# Autodesk Inventor assembly: вертикальный ЗАХВАТ
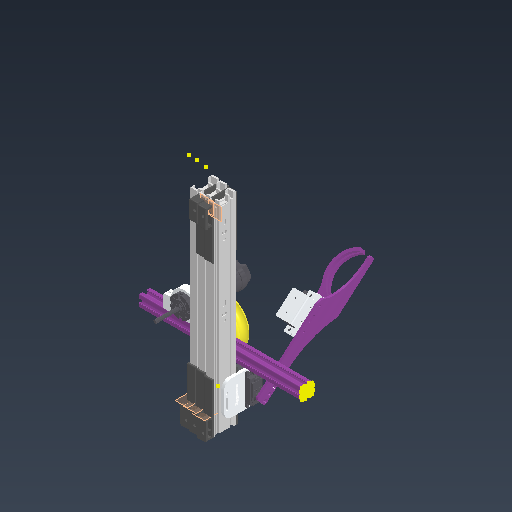
[picture p0: Inventor's stored thumbnail of the model, 512x512]
Saved by Autodesk Inventor 2025 (Build 290162000, 162)
## iProperties
Created: 2025-01-28
Part Number: вертикальный ЗАХВАТ
Document SubType Name: Assembly
Designer: GameHD
Author: GameHD
## Documents named in this file (12)
- C:\Users\GameHD\Desktop\phantom 16950\вертикальный ЗАХВАТ.iam
- C:\Users\GameHD\Desktop\phantom 16950\2000-0025-0002\2000-0025-0002_MIR1.ipt
- C:\Users\GameHD\Desktop\phantom 16950\клешня сос_MIR.ipt
- C:\Users\GameHD\Desktop\phantom 16950\39060_txm-standard servo bracket\39060_txm-standard servo bracket_MIR.ipt
- C:\Users\GameHD\Desktop\phantom 16950\Клешни с фиксатором\Клешни с фиксатором_MIR_MIR.ipt
- C:\Users\GameHD\Desktop\phantom 16950\профиль каркас ГОРИЗОНТ пенпер.ipt
- C:\Users\GameHD\Desktop\phantom 16950\35 напр.iam
- C:\Users\GameHD\Desktop\phantom 16950\39089_txm-motormount\39089_txm-motormount.ipt
- C:\Users\GameHD\Desktop\phantom 16950\REV-41-1211\REV-41-1211.ipt
- C:\Users\GameHD\Desktop\phantom 16950\пластинка для серв.ipt
- C:\Users\GameHD\Desktop\phantom 16950\katushechka_pushechka\katushechka_pushechka_CPY.ipt
- C:\Users\GameHD\Desktop\phantom 16950\katushechka_pushechka 2\katushechka_pushechka 2_CPY.ipt
## Components (12 placed, 11 different names)
1. профиль каркас ГОРИЗОНТ пенпер:1
2. 2000-0025-0002_MIR1:1
3. клешня сос_MIR:1
4. 39060_txm-standard servo bracket_MIR:1
5. 2000-0025-0002_MIR1:2
6. Клешни с фиксатором_MIR_MIR:1
7. 35 напр:1 [sub-assembly]
8. 39089_txm-motormount:1
9. REV-41-1211:1
10. пластинка для серв:1
11. katushechka_pushechka_CPY:1 — Совмещение:16, Совмещение:17
12. katushechka_pushechka 2_CPY:1 — Совмещение:16, Совмещение:17
## Relationships (19: Mate 14, Flush 5)
- [Flush] (-90 mm): клешня сос_MIR:1 ↔ 39060_txm-standard servo bracket_MIR:1
- [Flush]: клешня сос_MIR:1 ↔ 39060_txm-standard servo bracket_MIR:1
- [Mate]: клешня сос_MIR:1 ↔ 39060_txm-standard servo bracket_MIR:1
- [Mate] (4 mm): 39060_txm-standard servo bracket_MIR:1 ↔ 2000-0025-0002_MIR1:2
- [Flush] (2.5 mm): 39060_txm-standard servo bracket_MIR:1 ↔ 2000-0025-0002_MIR1:2
- [Mate]: 39060_txm-standard servo bracket_MIR:1 ↔ 2000-0025-0002_MIR1:2
- [Mate] (7 mm): клешня сос_MIR:1 ↔ Клешни с фиксатором_MIR_MIR:1
- [Mate]: 2000-0025-0002_MIR1:2 ↔ Клешни с фиксатором_MIR_MIR:1
- [Mate]: 2000-0025-0002_MIR1:2 ↔ Клешни с фиксатором_MIR_MIR:1
- [Mate]: профиль каркас ГОРИЗОНТ пенпер:1 ↔ 39089_txm-motormount:1
- [Flush]: профиль каркас ГОРИЗОНТ пенпер:1 ↔ 39089_txm-motormount:1
- [Mate]: 39089_txm-motormount:1 ↔ REV-41-1211:1
- [Mate]: 35 напр:1 ↔ пластинка для серв:1
- [Flush] (-16.2 mm): 35 напр:1 ↔ пластинка для серв:1
- [Mate] (1 mm): 2000-0025-0002_MIR1:1 ↔ пластинка для серв:1
- [Mate]: 2000-0025-0002_MIR1:1 ↔ пластинка для серв:1
- [Mate]: 2000-0025-0002_MIR1:1 ↔ пластинка для серв:1
- Совмещение:16 [Mate]: katushechka_pushechka_CPY:1 ↔ katushechka_pushechka 2_CPY:1
- Совмещение:17 [Mate]: katushechka_pushechka_CPY:1 ↔ katushechka_pushechka 2_CPY:1
